# Autodesk Inventor assembly: knee_w_motor
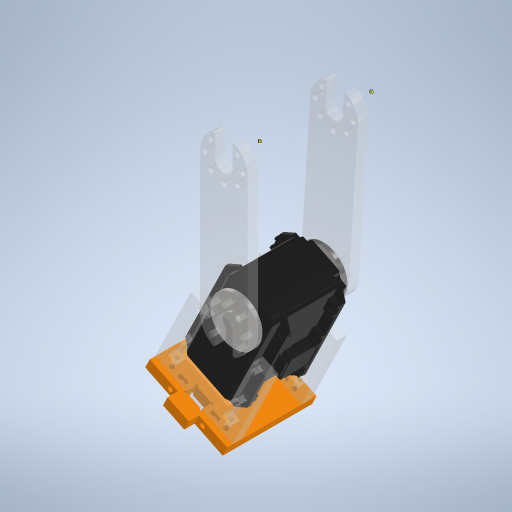
[picture p0: Inventor's stored thumbnail of the model, 512x512]
Saved by Autodesk Inventor 2024 (Build 280153000, 153)
## iProperties
Created: 2024-09-14
Part Number: knee_w_motor
Document SubType Name: Assembly
Designer: jmha0
Author: jmha0
## Documents named in this file (7)
- C:\Users\jmha0\OneDrive\바탕 화면\19th_intern_hjm_fight_robot\Lower_Body\knee_w_motor\knee_w_motor_fin1.iam
- C:\Users\jmha0\OneDrive\바탕 화면\19th_intern_hjm_fight_robot\Lower_Body\knee_w_motor\frame_ankle_to_knee1.ipt
- C:\Users\jmha0\OneDrive\바탕 화면\19th_intern_hjm_fight_robot\hardware\ROBOTIS(Inventor 2024 ver.)\다이나믹셀\MX-106T+idle.ipt.iam
- C:\Users\jmha0\OneDrive\바탕 화면\19th_intern_hjm_fight_robot\hardware\ROBOTIS(Inventor 2024 ver.)\혼\64-106Horn.ipt
- C:\Users\jmha0\OneDrive\바탕 화면\19th_intern_hjm_fight_robot\Lower_Body\knee_w_motor\frame_knee_to_bridge.ipt
- C:\Users\jmha0\OneDrive\바탕 화면\19th_intern_hjm_fight_robot\Lower_Body\knee_w_motor\bridge1.ipt
- MX-106T+idle.ipt
## Components (7 placed, 5 different names)
1. frame_ankle_to_knee1:1 — 삽입:3, 삽입:4, 삽입:5, 삽입:6, 삽입:10, 각도:1
2. MX-106T+idle.ipt:1 [sub-assembly] — 삽입:1, 삽입:11, 삽입:12, 삽입:13, 삽입:14, 삽입:15, 삽입:16, 삽입:17, 메이트:1
3. 64-106Horn:1 — 삽입:1, 삽입:3, 삽입:4, 삽입:5, 삽입:6, 삽입:10
4. frame_ankle_to_knee1:2 — 메이트:1, 각도:1
5. frame_knee_to_bridge:1 — 삽입:11, 삽입:12, 삽입:13, 삽입:19, 삽입:21
6. frame_knee_to_bridge:2 — 삽입:14, 삽입:15, 삽입:16, 삽입:17, 삽입:18, 삽입:20, 삽입:22
7. bridge1:1 — 삽입:18, 삽입:19, 삽입:20, 삽입:21, 삽입:22
## Relationships (20: Insert 18, Mate 1, Angle 1)
- 삽입:1 [Insert] (0.1 mm): MX-106T+idle.ipt:1 ↔ 64-106Horn:1
- 삽입:3 [Insert]: frame_ankle_to_knee1:1 ↔ 64-106Horn:1
- 삽입:4 [Insert]: frame_ankle_to_knee1:1 ↔ 64-106Horn:1
- 삽입:5 [Insert]: frame_ankle_to_knee1:1 ↔ 64-106Horn:1
- 삽입:6 [Insert]: frame_ankle_to_knee1:1 ↔ 64-106Horn:1
- 삽입:10 [Insert]: frame_ankle_to_knee1:1 ↔ 64-106Horn:1
- 삽입:11 [Insert]: MX-106T+idle.ipt:1 ↔ frame_knee_to_bridge:1
- 삽입:12 [Insert]: MX-106T+idle.ipt:1 ↔ frame_knee_to_bridge:1
- 삽입:13 [Insert]: MX-106T+idle.ipt:1 ↔ frame_knee_to_bridge:1
- 삽입:14 [Insert]: MX-106T+idle.ipt:1 ↔ frame_knee_to_bridge:2
- 삽입:15 [Insert]: MX-106T+idle.ipt:1 ↔ frame_knee_to_bridge:2
- 삽입:16 [Insert]: MX-106T+idle.ipt:1 ↔ frame_knee_to_bridge:2
- 삽입:17 [Insert]: MX-106T+idle.ipt:1 ↔ frame_knee_to_bridge:2
- 삽입:18 [Insert]: frame_knee_to_bridge:2 ↔ bridge1:1
- 삽입:19 [Insert]: frame_knee_to_bridge:1 ↔ bridge1:1
- 삽입:20 [Insert]: frame_knee_to_bridge:2 ↔ bridge1:1
- 삽입:21 [Insert]: frame_knee_to_bridge:1 ↔ bridge1:1
- 삽입:22 [Insert]: frame_knee_to_bridge:2 ↔ bridge1:1
- 메이트:1 [Mate]: MX-106T+idle.ipt:1 ↔ frame_ankle_to_knee1:2
- 각도:1 [Angle] (0 deg): frame_ankle_to_knee1:1 ↔ frame_ankle_to_knee1:2
